# Autodesk Inventor assembly: tester
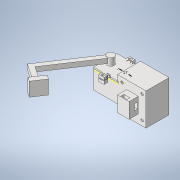
[picture p0: Inventor's stored thumbnail of the model, 180x180]
Saved by Autodesk Inventor 2020.2 (Build 242310000, 310)
## iProperties
Created: 2020-02-05
Part Number: tester
Document SubType Name: Assembly
Designer: ColinP
Author: ColinP
## Documents named in this file (5)
- C:\Users\ColinP\Documents\Inventor\steppermotoriqc\tester.iam
- C:\Users\ColinP\Documents\Inventor\steppermotoriqc\28BYJ-48 – 5V Stepper Motor\28BYJ-48 – 5V Stepper Motor.ipt
- C:\Users\ColinP\Documents\Inventor\steppermotoriqc\sheel.ipt
- C:\Users\ColinP\Documents\Inventor\steppermotoriqc\socket.ipt
- C:\Users\ColinP\Documents\Inventor\steppermotoriqc\shell 3.0.ipt
## Components (4 placed, 4 different names)
1. 28BYJ-48 – 5V Stepper Motor:1 — Mate:4, Mate:5, Tangent:2, Mate:6, Mate:7, Mate:10, Mate:11, Mate:12, Mate:13
2. sheel:1 — Mate:8, Mate:9, Mate:10
3. socket:1 — Mate:4, Mate:5, Tangent:2, Mate:6
4. shell 3.0:1 — Mate:7, Mate:8, Mate:9, Mate:11, Mate:12, Mate:13
## Relationships (11: Mate 10, Tangent 1)
- Mate:4: 28BYJ-48 – 5V Stepper Motor:1 ↔ socket:1
- Mate:5: 28BYJ-48 – 5V Stepper Motor:1 ↔ socket:1
- Tangent:2: 28BYJ-48 – 5V Stepper Motor:1 ↔ socket:1
- Mate:6: 28BYJ-48 – 5V Stepper Motor:1 ↔ socket:1
- Mate:7: 28BYJ-48 – 5V Stepper Motor:1 ↔ shell 3.0:1
- Mate:8: sheel:1 ↔ shell 3.0:1
- Mate:9: sheel:1 ↔ shell 3.0:1
- Mate:10: 28BYJ-48 – 5V Stepper Motor:1 ↔ sheel:1
- Mate:11: 28BYJ-48 – 5V Stepper Motor:1 ↔ shell 3.0:1
- Mate:12: 28BYJ-48 – 5V Stepper Motor:1 ↔ shell 3.0:1
- Mate:13: 28BYJ-48 – 5V Stepper Motor:1 ↔ shell 3.0:1
